# Autodesk Inventor assembly: Assembly1
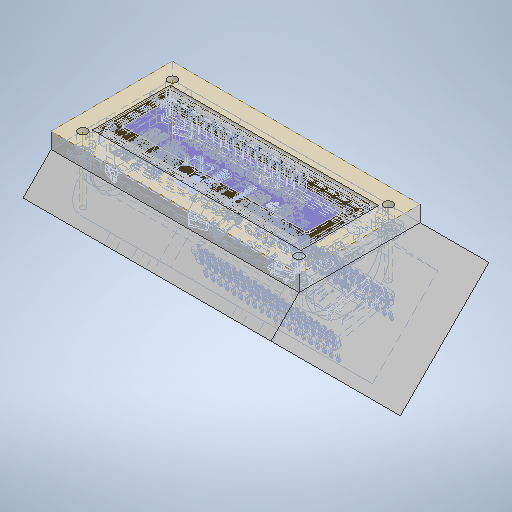
[picture p0: Inventor's stored thumbnail of the model, 512x512]
Saved by Autodesk Inventor 2025.2 (Build 292293000, 293)
## iProperties
Created: 2025-03-07
Part Number: Assembly1
Document SubType Name: Assembly
Designer: marye
Author: marye
## Documents named in this file (5)
- C:\Users\marye\OneDrive\Desktop\RhythmGuard\CAD\Assembly1.iam
- C:\Users\marye\Downloads\16x2 LCD Housing - 3839594\files\16x2_back_45deg_m2\16x2_back_45deg_m2\16x2_back_45deg_m2.ipt
- C:\Users\marye\Downloads\16-x-2-lcd-display-module-with-iic-i2c-module-1.snapshot.2\LCD AP214\LCD AP214\LCD AP214.ipt
- C:\Users\marye\Downloads\16x2 LCD Housing - 3839594\files\16x2_front_big_m3\16x2_front_big_m3\16x2_front_big_m3.ipt
- C:\Users\marye\Downloads\esp32-pico-kit-1.snapshot.5\ESP32-PICO-KIT\ESP32-PICO-KIT\ESP32-PICO-KIT.ipt
## Components (4 placed, 4 different names)
1. 16x2_back_45deg_m2:1 — Flush:2, Flush:3, Mate:3
2. LCD AP214:1 — Flush:1, Mate:1, Mate:2
3. 16x2_front_big_m3:1 — Flush:1, Mate:1, Mate:2, Flush:2, Flush:3, Mate:3
4. ESP32-PICO-KIT:1
## Relationships (6: Flush 3, Mate 3)
- Flush:1: LCD AP214:1 ↔ 16x2_front_big_m3:1
- Mate:1: LCD AP214:1 ↔ 16x2_front_big_m3:1
- Mate:2: LCD AP214:1 ↔ 16x2_front_big_m3:1
- Flush:2: 16x2_back_45deg_m2:1 ↔ 16x2_front_big_m3:1
- Flush:3: 16x2_back_45deg_m2:1 ↔ 16x2_front_big_m3:1
- Mate:3: 16x2_back_45deg_m2:1 ↔ 16x2_front_big_m3:1
